# Autodesk Inventor assembly: Вал в сборе
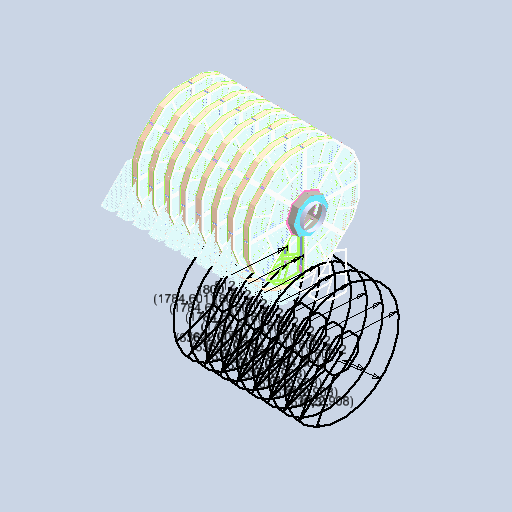
[picture p0: Inventor's stored thumbnail of the model, 512x512]
Saved by Autodesk Inventor 2024.2 (Build 282272000, 272)
## iProperties
Created: 2023-08-30
Part Number: Вал в сборе
Document SubType Name: Assembly
Designer: admin
Stock Number: Вал в сБоре
Author: admin
## Documents named in this file (3)
- C:\Users\pokla\Documents\Inventor\ДФО\Дисковый фильтр в инвенторе\New folder\Workspaces\Workspace\Вал в сборе\Вал в сборе.iam
- C:\Users\pokla\Documents\Inventor\ДФО\Дисковый фильтр в инвенторе\New folder\Workspaces\Workspace\Вал в сборе\îñíîâà áàðàáàíà.iam
- C:\Users\pokla\Documents\Inventor\ДФО\Дисковый фильтр в инвенторе\New folder\Workspaces\Workspace\Вал в сборе\фильтр-кольцо.iam
## Components (9 placed, 2 different names)
1. îñíîâà áàðàáàíà [sub-assembly] — Mate:1, Mate:2, Mate:3, Mate:4, Mate:5, Mate:6, Mate:7
2. фильтр-кольцо:1 [sub-assembly] — Mate:4, Mate:6, Mate:7
3. фильтр-кольцо:2 [sub-assembly]
4. фильтр-кольцо:3 [sub-assembly]
5. фильтр-кольцо:4 [sub-assembly]
6. фильтр-кольцо:5 [sub-assembly]
7. фильтр-кольцо:6 [sub-assembly]
8. фильтр-кольцо:7 [sub-assembly]
9. фильтр-кольцо:8 [sub-assembly]
## Component patterns: (8 elements, first: фильтр-кольцо:1)
## Relationships (7: Mate 7)
- Mate:1: îñíîâà áàðàáàíà
- Mate:2: îñíîâà áàðàáàíà
- Mate:3 (-1025 mm): îñíîâà áàðàáàíà
- Mate:4: îñíîâà áàðàáàíà ↔ фильтр-кольцо:1
- Mate:5: îñíîâà áàðàáàíà
- Mate:6: îñíîâà áàðàáàíà ↔ фильтр-кольцо:1
- Mate:7: îñíîâà áàðàáàíà ↔ фильтр-кольцо:1
